# Autodesk Inventor assembly: Dribbler_Type3
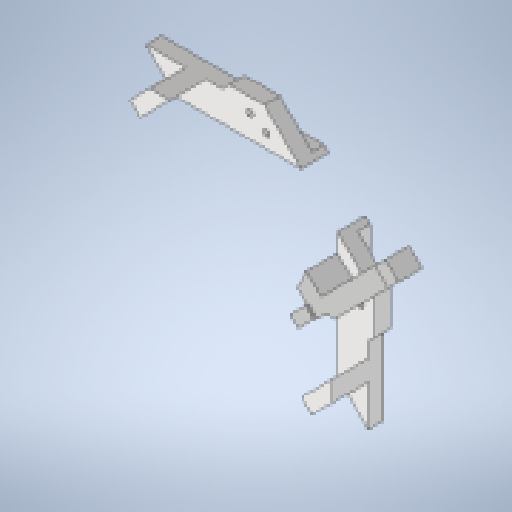
[picture p0: Inventor's stored thumbnail of the model, 512x512]
Saved by Autodesk Inventor 2025.1 (Build 291241000, 241)
## iProperties
Created: 2026-05-26
Part Number: Dribbler_Type3
Document SubType Name: Assembly
Designer: User
Author: User
## Documents named in this file (5)
- D:\One Drive\OneDrive - Politeknik Sultan Salahuddin Abdul Aziz Shah\Documents\Inventor\RobosotPSA\Dribbler_Type3.iam
- D:\One Drive\OneDrive - Politeknik Sultan Salahuddin Abdul Aziz Shah\Documents\Inventor\RobosotPSA\Dribbler_v3.ipt
- D:\One Drive\OneDrive - Politeknik Sultan Salahuddin Abdul Aziz Shah\Documents\Inventor\RobosotPSA\Drib_v3.ipt
- D:\One Drive\OneDrive - Politeknik Sultan Salahuddin Abdul Aziz Shah\Documents\Inventor\RobosotPSA\N20 Mini Micro Metall Gear Motor DC 3-6-12V v1\N20 Mini Micro Metall Gear Motor DC 3-6-12V v1\N20 Mini Micro Me.ipt
- D:\One Drive\OneDrive - Politeknik Sultan Salahuddin Abdul Aziz Shah\Documents\Inventor\RobosotPSA\Roller_Drib_v2.ipt
## Components (4 placed, 4 different names)
1. Drib_v3:1 — Mate:1, Mate:2, Mate:3, Mate:4, Mate:5, Flush:1
2. N20 Mini Micro Me:1 — Mate:1, Mate:2, Mate:3
3. Roller_Drib_v2:1 — Mate:4, Mate:5
4. Dribbler_v3:1 — Flush:1
## Relationships (6: Mate 5, Flush 1)
- Mate:1 (0.1 mm): Drib_v3:1 ↔ N20 Mini Micro Me:1
- Mate:2: Drib_v3:1 ↔ N20 Mini Micro Me:1
- Mate:3: Drib_v3:1 ↔ N20 Mini Micro Me:1
- Mate:4: Drib_v3:1 ↔ Roller_Drib_v2:1
- Mate:5 (2 mm): Drib_v3:1 ↔ Roller_Drib_v2:1
- Flush:1: Drib_v3:1 ↔ Dribbler_v3:1
